# Autodesk Inventor assembly: hips_assembly
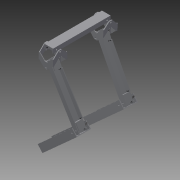
[picture p0: Inventor's stored thumbnail of the model, 180x180]
Saved by Autodesk Inventor 2015 (Build 190159000, 159)
## iProperties
Created: 2014-06-09
Part Number: hips_assembly
Document SubType Name: Assembly
Designer: L
Author: L
## Documents named in this file (3)
- C:\Users\Jaden\Documents\GitHub\SolidModels\stag_v2_01_pre_alpha\hips_assembly.iam
- C:\Users\Jaden\Documents\GitHub\SolidModels\stag_v2_01_pre_alpha\upper_leg.iam
- C:\Users\Jaden\Documents\GitHub\SolidModels\stag_v2_01_pre_alpha\leg_assembly.iam
## Components (3 placed, 2 different names)
1. upper_leg:1 [sub-assembly] — Mate:1, Mate:3, Flush:1, Mate:5, Mate:6, Angle:1, Mate:7, Angle:2
2. leg_assembly:1 [sub-assembly] — Mate:1, Mate:6, Angle:2
3. leg_assembly:2 [sub-assembly] — Mate:3, Angle:1, Mate:7
## Relationships (8: Mate 5, Angle 2, Flush 1)
- Mate:1: upper_leg:1 ↔ leg_assembly:1
- Mate:3: upper_leg:1 ↔ leg_assembly:2
- Flush:1: upper_leg:1
- Mate:5: upper_leg:1
- Mate:6: upper_leg:1 ↔ leg_assembly:1
- Angle:1 (0 deg): upper_leg:1 ↔ leg_assembly:2
- Mate:7: upper_leg:1 ↔ leg_assembly:2
- Angle:2 (180 deg): upper_leg:1 ↔ leg_assembly:1
